# Autodesk Inventor assembly: SmartCube
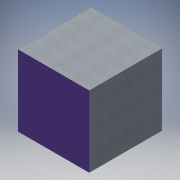
[picture p0: Inventor's stored thumbnail of the model, 180x180]
Saved by Autodesk Inventor 2018 (Build 220112000, 112)
## iProperties
Created: 2019-02-06
Part Number: SmartCube
Material: Generisch
Document SubType Name: Assembly
Designer: Lolob
Author: Lolob
## Documents named in this file (9)
- D:\Dokumente\S ch u l e\Dipl\Smartcube_Construction\Version_2\SmartCube_Quadratisch.iam
- D:\Dokumente\S ch u l e\Dipl\Smartcube_Construction\Version_2\Boden.ipt
- D:\Dokumente\S ch u l e\Dipl\Smartcube_Construction\Version_2\Wand1.ipt
- D:\Dokumente\S ch u l e\Dipl\Smartcube_Construction\Version_2\Wand1_MIR.ipt
- D:\Dokumente\S ch u l e\Dipl\Smartcube_Construction\Version_2\Wand2.ipt
- D:\Dokumente\S ch u l e\Dipl\Smartcube_Construction\Version_2\Wand2_MIR.ipt
- D:\Dokumente\S ch u l e\Dipl\Smartcube_Construction\Version_2\Baterie.ipt
- D:\Dokumente\Inventor\Projektname\PV_Modul.ipt
- D:\Dokumente\Inventor\Projektname\Sitzfläche.ipt
## Components (8 placed, 8 different names)
1. Boden:1 — Passend:1, Passend:2, Passend:3, Starr:1, Starr:2, Starr:4, Passend:7
2. Wand1:1 — Passend:1, Starr:1, Drehbar:1
3. Wand1_MIR:1 — Passend:2, Starr:4, Passend:11
4. Wand2:1 — Drehbar:1, Starr:5
5. Wand2_MIR:1 — Passend:3, Starr:2, Passend:11
6. Baterie:1 — Passend:7
7. PV_Modul:1 — Passend:9, Fluchtend:1, Passend:10
8. Sitzfläche:1 — Passend:9, Fluchtend:1, Passend:10, Starr:5
## Relationships (13: Mate 7, WeldJoint 4, RevoluteJoint 1, Flush 1)
- Passend:1 [Mate]: Boden:1 ↔ Wand1:1
- Passend:2 [Mate]: Boden:1 ↔ Wand1_MIR:1
- Passend:3 [Mate]: Boden:1 ↔ Wand2_MIR:1
- Starr:1 [WeldJoint]: Boden:1 ↔ Wand1:1
- Starr:2 [WeldJoint]: Boden:1 ↔ Wand2_MIR:1
- Starr:4 [WeldJoint]: Boden:1 ↔ Wand1_MIR:1
- Drehbar:1 [RevoluteJoint]: Wand1:1 ↔ Wand2:1
- Passend:7 [Mate]: Boden:1 ↔ Baterie:1
- Passend:9 [Mate]: PV_Modul:1 ↔ Sitzfläche:1
- Fluchtend:1 [Flush] (-10 mm): PV_Modul:1 ↔ Sitzfläche:1
- Passend:10 [Mate]: PV_Modul:1 ↔ Sitzfläche:1
- Starr:5 [WeldJoint]: Wand2:1 ↔ Sitzfläche:1
- Passend:11 [Mate]: Wand1_MIR:1 ↔ Wand2_MIR:1
